# Autodesk Inventor assembly: KS-14_SLow_10inch
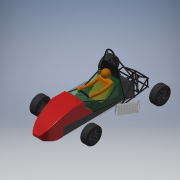
[picture p0: Inventor's stored thumbnail of the model, 180x180]
Saved by Autodesk Inventor 2018.1 (Build 221171000, 171)
## iProperties
Created: 2017-10-13
Part Number: KS-14_SLow_10inch
Material: 一般
Document SubType Name: Assembly
Designer: kuwano
Sending System: Autodesk Inventor 2018
Preprocessor: ST-DEVELOPER v16.13
Title: D:\kuwano\Documents\Inventor\KITformula\CFD_KS-14\KS-14\stl\final_assembly_2017_SuperUltraLow.stp
Author: kuwano
## Documents named in this file (11)
- D:\kuwano\Documents\Inventor\KITformula\KS-15_Aero_CAD\ks-14_slow\KS-14_SLow_10inch.iam
- D:\kuwano\Documents\Inventor\KITformula\KS-15_Aero_CAD\KS-14_SLow\parts\frame3kaiseki_retutch.ipt
- D:\kuwano\Documents\Inventor\KITformula\KS-15_Aero_CAD\KS-14_SLow\parts\driver.ipt
- D:\kuwano\Documents\Inventor\KITformula\KS-15_Aero_CAD\KS-14_SLow\parts\steering assembly.iam
- D:\kuwano\Documents\Inventor\KITformula\KS-15_Aero_CAD\KS-14_SLow\parts\2017 exhaust assembly_retouch.ipt
- D:\kuwano\Documents\Inventor\KITformula\KS-15_Aero_CAD\KS-14_SLow\parts\kaul_reretouch.ipt
- D:\kuwano\Documents\Inventor\KITformula\KS-15_Aero_CAD\KS-14_SLow\parts\newbody.ipt
- D:\kuwano\Documents\Inventor\KITformula\KS-15_Aero_CAD\KS-14_SLow\parts\radiator 2014 kaiseki.ipt
- D:\kuwano\Documents\Inventor\KITformula\KS-15_Aero_CAD\KS-14_SLow\parts\wall.ipt
- D:\kuwano\Documents\Inventor\KITformula\KS-15_Aero_CAD\KS-14_SLow\parts\wall_MIR1.ipt
- D:\kuwano\Documents\Inventor\KITformula\KS-15_Aero_CAD\ks-14_slow\parts\2015Wheel watanabe_10-13.ipt
## Components (13 placed, 10 different names)
1. frame3kaiseki_retutch:1 — メイト:2, メイト:3, メイト:4, メイト:5, メイト:6
2. driver:1
3. steering assembly:1 [sub-assembly]
4. 2017 exhaust assembly_retouch:1
5. kaul_reretouch:1 — メイト:1
6. newbody:1 — メイト:1
7. radiator 2014 kaiseki:1
8. wall:1 — フラッシュ:1, フラッシュ:2, フラッシュ:3, メイト:2, メイト:3, メイト:4, メイト:5, メイト:6
9. wall_MIR1:1 — メイト:7, メイト:8, フラッシュ:4
10. 2015Wheel watanabe_10-13:1
11. 2015Wheel watanabe_10-13:2
12. 2015Wheel watanabe_10-13:3
13. 2015Wheel watanabe_10-13:4
## Relationships (12: Mate 8, Flush 4)
- メイト:1 [Mate]: kaul_reretouch:1 ↔ newbody:1
- フラッシュ:1 [Flush]: wall:1
- フラッシュ:2 [Flush]: wall:1
- フラッシュ:3 [Flush]: wall:1
- メイト:2 [Mate]: frame3kaiseki_retutch:1 ↔ wall:1
- メイト:3 [Mate]: frame3kaiseki_retutch:1 ↔ wall:1
- メイト:4 [Mate]: frame3kaiseki_retutch:1 ↔ wall:1
- メイト:5 [Mate]: frame3kaiseki_retutch:1 ↔ wall:1
- メイト:6 [Mate]: frame3kaiseki_retutch:1 ↔ wall:1
- メイト:7 [Mate]: wall_MIR1:1
- メイト:8 [Mate]: wall_MIR1:1
- フラッシュ:4 [Flush]: wall_MIR1:1
